# Autodesk Inventor assembly: DoubleSlipHR_asmtest
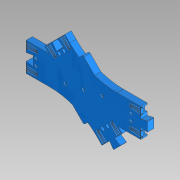
[picture p0: Inventor's stored thumbnail of the model, 180x180]
Saved by Autodesk Inventor 2021 (Build 250183000, 183)
## iProperties
Created: 2021-05-05
Part Number: DoubleSlipHR_asmtest
Document SubType Name: Assembly
Designer: kumagai
Author: kumagai
## Documents named in this file (7)
- X:\Develop\CAD\PlaRails\DoubleSlip\DoubleSlipHR_asmtest.iam
- X:\Develop\CAD\PlaRails\DoubleSlip\DoubleSlipHR_C.ipt
- X:\Develop\CAD\PlaRails\DoubleSlip\DoubleSlipHR_Bar.ipt
- X:\Develop\CAD\PlaRails\DoubleSlip\GearBarBase.ipt
- X:\Develop\CAD\PlaRails\DoubleSlip\GearCenter.ipt
- X:\Develop\CAD\PlaRails\DoubleSlip\GearCenterCover.ipt
- X:\Develop\CAD\PlaRails\DoubleSlip\DSHR_BarCover.ipt
## Components (7 placed, 6 different names)
1. DoubleSlipHR_C:1 — メイト:1, メイト:2, 回転:1, フラッシュ:1, メイト:3, メイト:4, メイト:5, フラッシュ:2, 回転:2
2. GearBarBase:1 — 回転:1
3. GearCenter:1 — 回転:2
4. GearCenterCover:1 — フラッシュ:1, メイト:3
5. DSHR_BarCover:1 — メイト:4, メイト:5, フラッシュ:2
6. DoubleSlipHR_Bar:1 — メイト:1, メイト:2
7. DoubleSlipHR_Bar:2
## Component patterns: (2 elements, first: DoubleSlipHR_Bar:1)
## Relationships (9: Mate 5, RevoluteJoint 2, Flush 2)
- メイト:1 [Mate]: DoubleSlipHR_C:1 ↔ DoubleSlipHR_Bar:1
- メイト:2 [Mate]: DoubleSlipHR_C:1 ↔ DoubleSlipHR_Bar:1
- 回転:1 [RevoluteJoint]: DoubleSlipHR_C:1 ↔ GearBarBase:1
- フラッシュ:1 [Flush]: DoubleSlipHR_C:1 ↔ GearCenterCover:1
- メイト:3 [Mate]: DoubleSlipHR_C:1 ↔ GearCenterCover:1
- メイト:4 [Mate]: DoubleSlipHR_C:1 ↔ DSHR_BarCover:1
- メイト:5 [Mate]: DoubleSlipHR_C:1 ↔ DSHR_BarCover:1
- フラッシュ:2 [Flush]: DoubleSlipHR_C:1 ↔ DSHR_BarCover:1
- 回転:2 [RevoluteJoint]: DoubleSlipHR_C:1 ↔ GearCenter:1
